# Autodesk Inventor assembly: Assem1
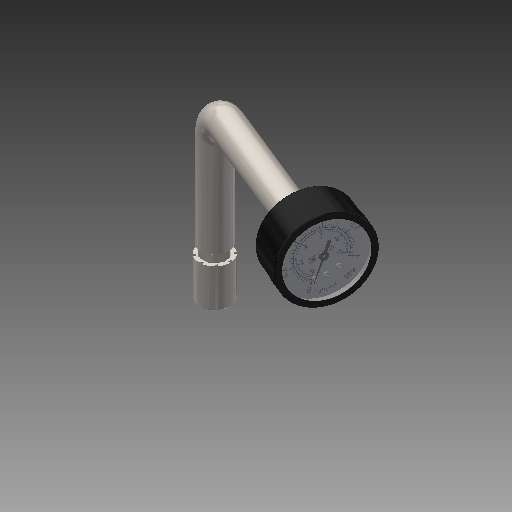
[picture p0: Inventor's stored thumbnail of the model, 512x512]
Saved by Autodesk Inventor 2017 (Build 210142000, 142)
## iProperties
Created: 2014-08-02
Part Number: Assem1
Document SubType Name: Assembly
Designer: XuZhiqing
Author: XuZhiqing
## Documents named in this file (6)
- C:\Users\XuZhiqing\Desktop\Project01-CFD_the_sys\CAD-Whole Sys v1.02\filter and gauge\filter and gauge\pressure gauge.iam
- C:\Users\XuZhiqing\Desktop\Project01-CFD_the_sys\CAD-Whole Sys v1.02\filter and gauge\filter and gauge\Part10.ipt
- C:\Users\XuZhiqing\Desktop\Project01-CFD_the_sys\CAD-Whole Sys v1.02\filter and gauge\filter and gauge\Part19.ipt
- C:\Users\XuZhiqing\Desktop\Project01-CFD_the_sys\CAD-Whole Sys v1.02\filter and gauge\filter and gauge\Part21.ipt
- C:\Users\XuZhiqing\Desktop\Project01-CFD_the_sys\CAD-Whole Sys v1.02\filter and gauge\filter and gauge\gauge3.ipt
- C:\Users\XuZhiqing\Desktop\Project01-CFD_the_sys\CAD-Whole Sys v1.02\filter and gauge\filter and gauge\Solid9.ipt
## Components (6 placed, 5 different names)
1. Part10:1 — Mate:2, Mate:3, Mate:4, Mate:5
2. Part19:1 — Mate:4, Mate:5, Mate:7, Mate:8
3. Part21:1 — Mate:2, Mate:3
4. gauge3:1 — Mate:9
5. Solid9:1
6. Part10:2 — Mate:7, Mate:8, Mate:9
## Relationships (7: Mate 7)
- Mate:2: Part10:1 ↔ Part21:1
- Mate:3: Part10:1 ↔ Part21:1
- Mate:4: Part10:1 ↔ Part19:1
- Mate:5: Part10:1 ↔ Part19:1
- Mate:7: Part19:1 ↔ Part10:2
- Mate:8: Part19:1 ↔ Part10:2
- Mate:9: gauge3:1 ↔ Part10:2
